# Autodesk Inventor assembly: Assembly2
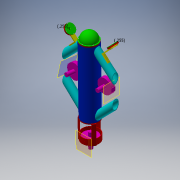
[picture p0: Inventor's stored thumbnail of the model, 180x180]
Saved by Autodesk Inventor 2016 (Build 200138000, 138)
## iProperties
Created: 2017-09-28
Part Number: Assembly2
Document SubType Name: Assembly
Designer: Student
Author: Student
## Documents named in this file (9)
- C:\Users\Student\Documents\Derek Code and Projects\ROV V2\Assembly2.iam
- C:\Users\Student\Documents\Derek Code and Projects\ROV V2\Angled Pipe (Attached to Control Pipe).ipt
- C:\Users\Student\Documents\Derek Code and Projects\ROV V2\Control Pipe V2.ipt
- C:\Users\Student\Documents\Derek Code and Projects\CodeBenderCode-master\ROV CAD Electronics\T100 rough draft.ipt
- C:\Users\Student\Documents\Derek Code and Projects\Autodesk\LED housing Assembly.iam
- C:\Users\Student\Documents\Derek Code and Projects\CodeBenderCode-master\ROV Prototype CAD Models FAILS\O ring Dome 2.ipt
- C:\Users\Student\Documents\Derek Code and Projects\CodeBenderCode-master\ROV Prototype CAD Models FAILS\ROV Dome 4'' (1).0004.ipt
- C:\Users\Student\Documents\Inventor\Content Center Files\R2016\en-US\BS 4183(7)\BS 4183 - M3.5 x 5(2) III.ipt
- C:\Users\Student\Documents\Derek Code and Projects\ROV V2\O ring fitting with motor mount.ipt
## Components (19 placed, 8 different names)
1. Angled Pipe (Attached to Control Pipe):3 — Mate:2, Mate:7, Mate:16
2. Angled Pipe (Attached to Control Pipe):4 — Mate:1, Mate:16
3. Control Pipe V2:1 — Mate:1, Mate:2, Mate:3, Mate:4, Mate:5, Mate:8, Mate:9, Mate:10, Mate:13, Mate:14
4. Angled Pipe (Attached to Control Pipe):5 — Mate:4, Mate:6, Mate:15
5. Angled Pipe (Attached to Control Pipe):6 — Mate:3, Mate:15
6. T100 rough draft:2
7. T100 rough draft:3
8. T100 rough draft:4 — Mate:5
9. LED housing Assembly:1 [sub-assembly] — Mate:6
10. LED housing Assembly:2 [sub-assembly] — Mate:7
11. O ring Dome 2:1 — Mate:8, Mate:9, Mate:11, Mate:12
12. ROV Dome 4'' (1).0004:1 — Mate:10, Mate:11, Mate:12, Insert:1, Insert:2, Insert:3, Insert:4, Insert:5, Insert:6
13. BS 4183 Slotted Pan Head Machine Screw - Metric M3.5 x 5:1 — Insert:1
14. BS 4183 Slotted Pan Head Machine Screw - Metric M3.5 x 5:2 — Insert:2
15. BS 4183 Slotted Pan Head Machine Screw - Metric M3.5 x 5:3 — Insert:3
16. BS 4183 Slotted Pan Head Machine Screw - Metric M3.5 x 5:4 — Insert:4
17. BS 4183 Slotted Pan Head Machine Screw - Metric M3.5 x 5:5 — Insert:5
18. BS 4183 Slotted Pan Head Machine Screw - Metric M3.5 x 5:6 — Insert:6
19. O ring fitting with motor mount:1 — Mate:13, Mate:14
## Relationships (22: Mate 16, Insert 6)
- Mate:1: Angled Pipe (Attached to Control Pipe):4 ↔ Control Pipe V2:1
- Mate:2: Angled Pipe (Attached to Control Pipe):3 ↔ Control Pipe V2:1
- Mate:3: Control Pipe V2:1 ↔ Angled Pipe (Attached to Control Pipe):6
- Mate:4: Control Pipe V2:1 ↔ Angled Pipe (Attached to Control Pipe):5
- Mate:5: Control Pipe V2:1 ↔ T100 rough draft:4
- Mate:6 (19.05 mm): Angled Pipe (Attached to Control Pipe):5 ↔ LED housing Assembly:1
- Mate:7 (19.05 mm): Angled Pipe (Attached to Control Pipe):3 ↔ LED housing Assembly:2
- Mate:8: Control Pipe V2:1 ↔ O ring Dome 2:1
- Mate:9: Control Pipe V2:1 ↔ O ring Dome 2:1
- Mate:10: Control Pipe V2:1 ↔ ROV Dome 4'' (1).0004:1
- Mate:11: O ring Dome 2:1 ↔ ROV Dome 4'' (1).0004:1
- Mate:12: O ring Dome 2:1 ↔ ROV Dome 4'' (1).0004:1
- Insert:1: ROV Dome 4'' (1).0004:1 ↔ BS 4183 Slotted Pan Head Machine Screw - Metric M3.5 x 5:1
- Insert:2: ROV Dome 4'' (1).0004:1 ↔ BS 4183 Slotted Pan Head Machine Screw - Metric M3.5 x 5:2
- Insert:3: ROV Dome 4'' (1).0004:1 ↔ BS 4183 Slotted Pan Head Machine Screw - Metric M3.5 x 5:3
- Insert:4: ROV Dome 4'' (1).0004:1 ↔ BS 4183 Slotted Pan Head Machine Screw - Metric M3.5 x 5:4
- Insert:5: ROV Dome 4'' (1).0004:1 ↔ BS 4183 Slotted Pan Head Machine Screw - Metric M3.5 x 5:5
- Insert:6: ROV Dome 4'' (1).0004:1 ↔ BS 4183 Slotted Pan Head Machine Screw - Metric M3.5 x 5:6
- Mate:13: Control Pipe V2:1 ↔ O ring fitting with motor mount:1
- Mate:14: Control Pipe V2:1 ↔ O ring fitting with motor mount:1
- Mate:15: Angled Pipe (Attached to Control Pipe):5 ↔ Angled Pipe (Attached to Control Pipe):6
- Mate:16: Angled Pipe (Attached to Control Pipe):3 ↔ Angled Pipe (Attached to Control Pipe):4
